# Autodesk Inventor assembly: White Pawn
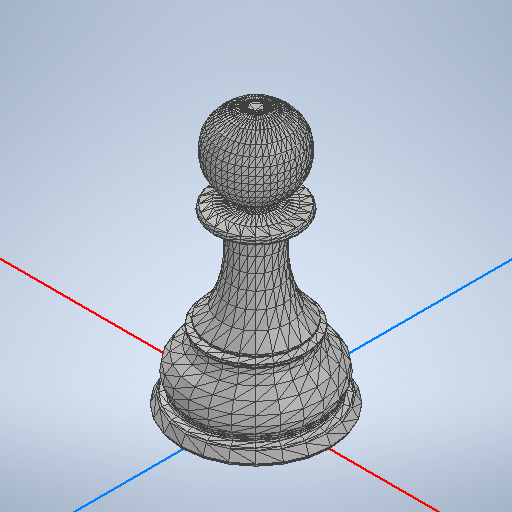
[picture p0: Inventor's stored thumbnail of the model, 512x512]
Saved by Autodesk Inventor 2025.2 (Build 292293000, 293)
## iProperties
Created: 2025-04-15
Part Number: White Pawn
Document SubType Name: Assembly
Designer: ckyiu
Author: ckyiu
## Documents named in this file (3)
- F:\Chessboard-Design\design\Assemblies\Chess Pieces\White Pawn.iam
- F:\Chessboard-Design\design\Parts\Chess Pieces\White Pawn.ipt
- F:\Chessboard-Design\design\Parts\Generic Neodynium Magnet 10mm diameter 2mm height.ipt
## Components (2 placed, 2 different names)
1. White Pawn:1 — Insert:1
2. Generic Neodynium Magnet 10mm diameter 2mm height:1 — Insert:1
## Relationships (1: Insert 1)
- Insert:1: White Pawn:1 ↔ Generic Neodynium Magnet 10mm diameter 2mm height:1
